# Autodesk Inventor assembly: JukeBox
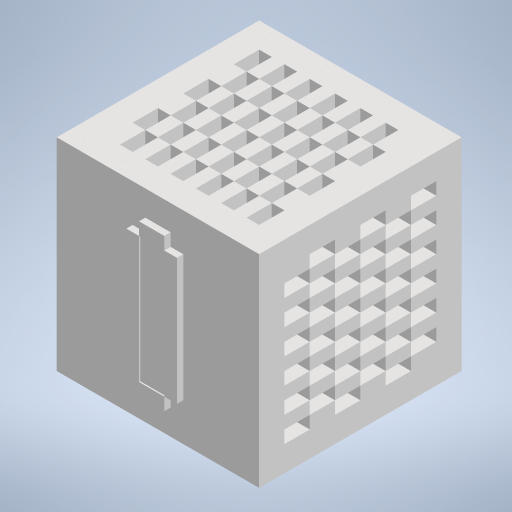
[picture p0: Inventor's stored thumbnail of the model, 512x512]
Saved by Autodesk Inventor 2024 (Build 280153000, 153)
## iProperties
Created: 2023-04-26
Part Number: JukeBox
Document SubType Name: Assembly
Designer: newic
Author: newic
## Documents named in this file (6)
- D:\My Models\JukeBox.iam
- D:\My Models\JukeBox Metal Frame.ipt
- D:\My Models\JukeBox CD Player.ipt
- D:\My Models\JukeBox Outside panel sharp edges.ipt
- D:\My Models\JukeBox Bottem Panel.ipt
- D:\My Models\JukeBox Top Panel.ipt
## Components (8 placed, 5 different names)
1. JukeBox Metal Frame:1 — Mate:1, Mate:2, Mate:3, Mate:4, Mate:5, Mate:6, Mate:7, Mate:8, Mate:9, Mate:10, Mate:11, Mate:12, Flush:1, Flush:2, Flush:3, Flush:4, Flush:5, Flush:6
2. JukeBox CD Player:1 — Mate:13, Mate:14, Mate:15
3. JukeBox Outside panel sharp edges:1 — Mate:3, Mate:4, Flush:2
4. JukeBox Outside panel sharp edges:2 — Mate:7, Mate:8, Flush:4
5. JukeBox Outside panel sharp edges:3 — Mate:5, Mate:6, Flush:3
6. JukeBox Outside panel sharp edges:4 — Mate:9, Mate:10, Flush:1
7. JukeBox Bottem Panel:1 — Mate:11, Mate:12, Flush:5, Mate:15
8. JukeBox Top Panel:1 — Mate:1, Mate:2, Flush:6, Mate:13, Mate:14
## Relationships (21: Mate 15, Flush 6)
- Mate:1: JukeBox Metal Frame:1 ↔ JukeBox Top Panel:1
- Mate:2: JukeBox Metal Frame:1 ↔ JukeBox Top Panel:1
- Mate:3: JukeBox Metal Frame:1 ↔ JukeBox Outside panel sharp edges:1
- Mate:4: JukeBox Metal Frame:1 ↔ JukeBox Outside panel sharp edges:1
- Mate:5: JukeBox Metal Frame:1 ↔ JukeBox Outside panel sharp edges:3
- Mate:6: JukeBox Metal Frame:1 ↔ JukeBox Outside panel sharp edges:3
- Mate:7: JukeBox Metal Frame:1 ↔ JukeBox Outside panel sharp edges:2
- Mate:8: JukeBox Metal Frame:1 ↔ JukeBox Outside panel sharp edges:2
- Mate:9: JukeBox Metal Frame:1 ↔ JukeBox Outside panel sharp edges:4
- Mate:10: JukeBox Metal Frame:1 ↔ JukeBox Outside panel sharp edges:4
- Mate:11: JukeBox Metal Frame:1 ↔ JukeBox Bottem Panel:1
- Mate:12: JukeBox Metal Frame:1 ↔ JukeBox Bottem Panel:1
- Flush:1: JukeBox Metal Frame:1 ↔ JukeBox Outside panel sharp edges:4
- Flush:2: JukeBox Metal Frame:1 ↔ JukeBox Outside panel sharp edges:1
- Flush:3: JukeBox Metal Frame:1 ↔ JukeBox Outside panel sharp edges:3
- Flush:4: JukeBox Metal Frame:1 ↔ JukeBox Outside panel sharp edges:2
- Flush:5: JukeBox Metal Frame:1 ↔ JukeBox Bottem Panel:1
- Flush:6: JukeBox Metal Frame:1 ↔ JukeBox Top Panel:1
- Mate:13: JukeBox CD Player:1 ↔ JukeBox Top Panel:1
- Mate:14: JukeBox CD Player:1 ↔ JukeBox Top Panel:1
- Mate:15: JukeBox CD Player:1 ↔ JukeBox Bottem Panel:1
